# Autodesk Inventor assembly: marco
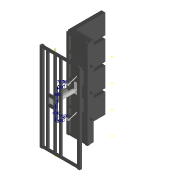
[picture p0: Inventor's stored thumbnail of the model, 180x180]
Saved by Autodesk Inventor 2021 (Build 250183000, 183)
## iProperties
Created: 2021-04-11
Part Number: marco
Document SubType Name: Assembly
Designer: equip
Mass: 593461 g
Surface Area: 184021 cm^2
Volume: 307399 cm^3
Density: 1.93059 g/cm^3
_SolveAssemblyDoc: Frame Generator Solve Assembly
_Version: 25.0.0
Author: equip
## Documents named in this file (12)
- C:\Users\Santiago Suárez\Documents\GitHub\Dis.-Mecatronico-E6\inventor proyecto\marco.iam
- C:\Users\Santiago Suárez\Documents\GitHub\Dis.-Mecatronico-E6\inventor proyecto\placa centro.ipt
- C:\Users\Santiago Suárez\Documents\GitHub\Dis.-Mecatronico-E6\inventor proyecto\Silla del marco.ipt
- C:\Users\Santiago Suárez\Documents\GitHub\Dis.-Mecatronico-E6\inventor proyecto\cilindro\cilindro.iam
- C:\Users\Santiago Suárez\Documents\GitHub\Dis.-Mecatronico-E6\inventor proyecto\marco inferior.ipt
- C:\Users\Santiago Suárez\Documents\GitHub\Dis.-Mecatronico-E6\inventor proyecto\marco\Frame\Marco Inferior.iam
- C:\Users\Santiago Suárez\Documents\GitHub\Dis.-Mecatronico-E6\inventor proyecto\MarcoSuperior.iam
- C:\Users\Santiago Suárez\Documents\GitHub\Dis.-Mecatronico-E6\inventor proyecto\Motor1.ipt
- C:\Users\Santiago Suárez\Documents\GitHub\Dis.-Mecatronico-E6\inventor proyecto\PlacaInferior.ipt
- C:\Users\Santiago Suárez\Documents\GitHub\Dis.-Mecatronico-E6\inventor proyecto\Eje.ipt
- C:\Users\Santiago Suárez\Documents\GitHub\Dis.-Mecatronico-E6\inventor proyecto\manivela.ipt
- C:\Users\Santiago Suárez\Documents\GitHub\Dis.-Mecatronico-E6\inventor proyecto\Biela.iam
## Components (17 placed, 11 different names)
1. placa centro:1 — Rigid:3, Rigid:11
2. marco inferior:1
3. Marco Inferior:1 [sub-assembly] — Mate:23, Mate:24
4. MarcoSuperior:1 [sub-assembly] — Rigid:3, Mate:21, Mate:22, Mate:28, Mate:29, Mate:30, Mate:32, Mate:33, Mate:34
5. PlacaInferior:1 — Mate:23, Mate:24, Mate:25, Mate:26, Mate:27, Rigid:12
6. cilindro:1 [sub-assembly] — Mate:25, Mate:26, Mate:27, Rigid:11
7. Motor1:1 — Rigid:12, Rotational:1, Rotational:2
8. Eje:1 — Rotational:1, Rigid:13
9. Eje:2 — Rotational:2, Rigid:14
10. manivela:1 — Rigid:13, Rigid:15
11. manivela:2 — Rigid:14, Rigid:16
12. Biela:1 [sub-assembly] — Rigid:15, Mate:28, Mate:29, Mate:30
13. Biela:2 [sub-assembly] — Rigid:16, Mate:32, Mate:33, Mate:34
14. Silla del marco:1 — Mate:21, Mate:22
15. Silla del marco:2
16. Silla del marco:3
17. Silla del marco:4
## Component patterns: (4 elements, first: Silla del marco:1)
## Relationships (22: Mate 13, WeldJoint 7, RevoluteJoint 2)
- Rigid:3 [WeldJoint]: placa centro:1 ↔ MarcoSuperior:1
- Mate:21 (-10 mm): MarcoSuperior:1 ↔ Silla del marco:1
- Mate:22: MarcoSuperior:1 ↔ Silla del marco:1
- Mate:23: Marco Inferior:1 ↔ PlacaInferior:1
- Mate:24: Marco Inferior:1 ↔ PlacaInferior:1
- Mate:25: PlacaInferior:1 ↔ cilindro:1
- Mate:26 (88.5 mm): PlacaInferior:1 ↔ cilindro:1
- Mate:27 (-100 mm): PlacaInferior:1 ↔ cilindro:1
- Rigid:11 [WeldJoint]: placa centro:1 ↔ cilindro:1
- Rigid:12 [WeldJoint]: PlacaInferior:1 ↔ Motor1:1
- Rotational:1 [RevoluteJoint]: Motor1:1 ↔ Eje:1
- Rotational:2 [RevoluteJoint]: Motor1:1 ↔ Eje:2
- Rigid:13 [WeldJoint]: Eje:1 ↔ manivela:1
- Rigid:14 [WeldJoint]: Eje:2 ↔ manivela:2
- Rigid:15 [WeldJoint] (-4 mm): manivela:1 ↔ Biela:1
- Rigid:16 [WeldJoint] (-4 mm): manivela:2 ↔ Biela:2
- Mate:28: MarcoSuperior:1 ↔ Biela:1
- Mate:29 (257.5 mm): MarcoSuperior:1 ↔ Biela:1
- Mate:30 (8 mm): MarcoSuperior:1 ↔ Biela:1
- Mate:32 (257.5 mm): MarcoSuperior:1 ↔ Biela:2
- Mate:33: MarcoSuperior:1 ↔ Biela:2
- Mate:34 (8 mm): MarcoSuperior:1 ↔ Biela:2
## Named parameters: sa_0 = 470880, sa_1 = 470880, sa_2 = 470880, sa_3 = 470880, sa_4 = 1000, sa_5 = 1e+06, sa_6 = 1e+06
note: some values were not read from the file. Shown as the stored number, unit unknown: "sa_0", "sa_1", "sa_2", "sa_3", "sa_4", "sa_5", "sa_6".
